# Autodesk Inventor assembly: brazo robot
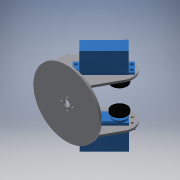
[picture p0: Inventor's stored thumbnail of the model, 180x180]
Saved by Autodesk Inventor 2018 (Build 220112000, 112)
## iProperties
Created: 2020-03-10
Part Number: brazo robot
Material: Genérico
Document SubType Name: Assembly
Designer: sala.ceri
Author: sala.ceri
## Documents named in this file (5)
- C:\Users\david\OneDrive\Documents\robot\ensamble\part2.iam
- C:\Users\david\OneDrive\Documents\robot\base.ipt
- C:\Users\david\OneDrive\Documents\robot\hombro.ipt
- C:\Users\david\OneDrive\Documents\robot\piezas\ServoMotor.ipt
- C:\Users\david\OneDrive\Documents\robot\piezas\BaseServo.ipt
## Components (7 placed, 4 different names)
1. base:1 — Coincidencia:11, Coincidencia:12, Coincidencia:13, Coincidencia:14
2. hombro:1 — Coincidencia:5, Coincidencia:7, Coincidencia:11, Coincidencia:12
3. hombro:2 — Coincidencia:6, Coincidencia:8, Coincidencia:9, Coincidencia:10, Coincidencia:13, Coincidencia:14
4. ServoMotor:1 — Coincidencia:8, Coincidencia:9, Coincidencia:10, Coincidencia:15, Coincidencia:23, Coincidencia:24
5. ServoMotor:2 — Coincidencia:5, Coincidencia:6, Coincidencia:7, Coincidencia:16
6. BaseServo:1 — Coincidencia:15, Coincidencia:16
7. BaseServo:2 — Coincidencia:23, Coincidencia:24
## Relationships (14: Mate 14)
- Coincidencia:5 [Mate]: hombro:1 ↔ ServoMotor:2
- Coincidencia:6 [Mate]: hombro:2 ↔ ServoMotor:2
- Coincidencia:7 [Mate]: hombro:1 ↔ ServoMotor:2
- Coincidencia:8 [Mate]: hombro:2 ↔ ServoMotor:1
- Coincidencia:9 [Mate]: hombro:2 ↔ ServoMotor:1
- Coincidencia:10 [Mate]: hombro:2 ↔ ServoMotor:1
- Coincidencia:11 [Mate]: base:1 ↔ hombro:1
- Coincidencia:12 [Mate]: base:1 ↔ hombro:1
- Coincidencia:13 [Mate]: base:1 ↔ hombro:2
- Coincidencia:14 [Mate]: base:1 ↔ hombro:2
- Coincidencia:15 [Mate]: ServoMotor:1 ↔ BaseServo:1
- Coincidencia:16 [Mate]: ServoMotor:2 ↔ BaseServo:1
- Coincidencia:23 [Mate]: ServoMotor:1 ↔ BaseServo:2
- Coincidencia:24 [Mate]: ServoMotor:1 ↔ BaseServo:2
